# Autodesk Inventor assembly: RT_FRM_A_003_Frame
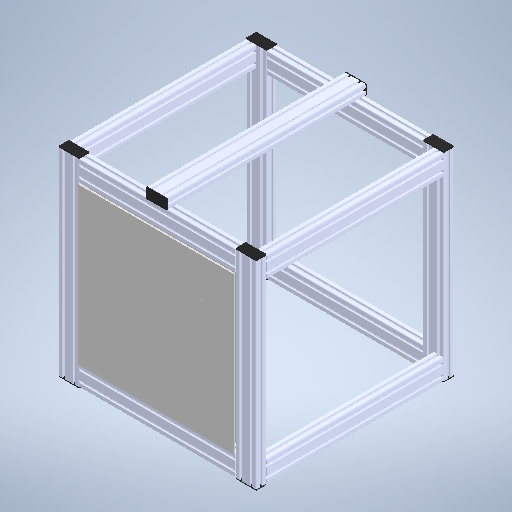
[picture p0: Inventor's stored thumbnail of the model, 512x512]
Saved by Autodesk Inventor 2025.4 (Build 294407000, 407)
## iProperties
Created: 2026-05-11
Part Number: RT_FRM_A_003_Frame
Document SubType Name: Assembly
Designer: louis
Author: louis
## Documents named in this file (7)
- C:\Users\louis\OneDrive\Desktop\R_Trident\02_CAD\04_Subassemblies\RT_FRM_A_003_Frame.iam
- C:\Users\louis\OneDrive\Desktop\R_Trident\02_CAD\01_Standard_Parts\Aluminium_Extrusions\4080x600_3620_2025012844725.ipt
- C:\Users\louis\OneDrive\Desktop\R_Trident\02_CAD\01_Standard_Parts\Aluminium_Extrusions\4080x680_3620_2025012844725.ipt
- C:\Users\louis\OneDrive\Desktop\R_Trident\02_CAD\01_Standard_Parts\Aluminium_Extrusions\4080x760_3620_2025012844725.ipt
- C:\Users\louis\OneDrive\Desktop\R_Trident\02_CAD\01_Standard_Parts\Aluminium_Extrusions\4080-cover.ipt
- C:\Users\louis\OneDrive\Desktop\R_Trident\02_CAD\03_Parts_Custom\RT_FRM_MC_009_ElectricalBackPlate.ipt
- C:\Users\louis\OneDrive\Desktop\R_Trident\02_CAD\03_Parts_Custom\RT_FRM_MC_009_ElectricalBackPlate_Inside.ipt
## Components (28 placed, 6 different names)
1. RT_FRM_MC_009_ElectricalBackPlate:1 — Mate:50, Mate:51, Mate:52
2. RT_FRM_MC_009_ElectricalBackPlate_Inside:1 — Mate:48, Mate:49, Flush:48
3. 4080x680_3620_2025012844725:4 — Mate:10, Mate:11, Flush:14
4. 4080x680_3620_2025012844725:3 — Mate:15, Mate:16, Flush:19
5. 4080x680_3620_2025012844725:2 — Flush:15, Mate:12, Mate:13
6. 4080x680_3620_2025012844725:1 — Mate:17, Mate:18, Flush:20
7. 4080x600_3620_2025012844725:4 — Flush:13, Mate:6, Mate:7
8. 4080x600_3620_2025012844725:3 — Flush:12, Mate:8, Mate:9
9. 4080x600_3620_2025012844725:2 — Mate:4, Mate:5, Flush:11, Mate:50, Mate:52
10. 4080x600_3620_2025012844725:1 — Mate:1, Mate:2, Flush:10, Mate:3, Mate:19, Mate:20, Flush:21, Flush:22, Mate:49, Flush:48
11. 4080x760_3620_2025012844725:5 — Mate:19, Flush:21, Mate:37, Mate:38, Mate:43, Mate:44, Mate:45
12. 4080-cover:6 — Mate:37, Mate:38
13. 4080-cover:11 — Mate:43, Mate:44
14. 4080x760_3620_2025012844725:6 — Mate:20, Flush:22, Mate:39, Mate:40, Mate:41, Mate:42
15. 4080-cover:7 — Mate:39, Mate:40
16. 4080-cover:9 — Mate:41, Mate:42
17. 4080x760_3620_2025012844725:1 — Flush:1, Flush:6, Flush:8, Mate:3, Mate:5, Mate:10, Mate:13, Flush:17, Mate:23, Mate:24, Mate:29, Mate:30, Mate:51
18. 4080-cover:1 — Mate:23, Mate:24
19. 4080-cover:12 — Mate:29, Mate:30
20. 4080x760_3620_2025012844725:2 — Flush:3, Flush:5, Flush:9, Flush:12, Mate:7, Mate:8, Mate:16, Flush:19, Mate:17, Mate:27, Mate:28, Mate:33, Mate:34
21. 4080-cover:5 — Mate:33, Mate:34
22. 4080-cover:10 — Mate:27, Mate:28
23. 4080x760_3620_2025012844725:3 — Flush:2, Flush:6, Flush:9, Flush:13, Mate:6, Mate:9, Mate:11, Flush:14, Flush:15, Mate:12, Flush:16, Mate:25, Mate:26, Mate:35, Mate:36
24. 4080-cover:2 — Mate:35, Mate:36
25. 4080-cover:8 — Mate:25, Mate:26
26. 4080x760_3620_2025012844725:4 — Flush:4, Flush:5, Flush:8, Mate:1, Mate:2, Flush:10, Mate:4, Flush:11, Mate:15, Mate:18, Flush:20, Mate:21, Mate:22, Mate:31, Mate:32, Mate:48
27. 4080-cover:3 — Mate:21, Mate:22
28. 4080-cover:4 — Mate:31, Mate:32
## Relationships (72: Mate 50, Flush 22)
- Flush:1: 4080x760_3620_2025012844725:1
- Flush:2: 4080x760_3620_2025012844725:3
- Flush:3: 4080x760_3620_2025012844725:2
- Flush:4: 4080x760_3620_2025012844725:4
- Flush:5: 4080x760_3620_2025012844725:2 ↔ 4080x760_3620_2025012844725:4
- Flush:6: 4080x760_3620_2025012844725:1 ↔ 4080x760_3620_2025012844725:3
- Flush:8: 4080x760_3620_2025012844725:1 ↔ 4080x760_3620_2025012844725:4
- Flush:9: 4080x760_3620_2025012844725:2 ↔ 4080x760_3620_2025012844725:3
- Mate:1: 4080x600_3620_2025012844725:1 ↔ 4080x760_3620_2025012844725:4
- Mate:2: 4080x600_3620_2025012844725:1 ↔ 4080x760_3620_2025012844725:4
- Flush:10: 4080x600_3620_2025012844725:1 ↔ 4080x760_3620_2025012844725:4
- Mate:3: 4080x600_3620_2025012844725:1 ↔ 4080x760_3620_2025012844725:1
- Mate:4: 4080x600_3620_2025012844725:2 ↔ 4080x760_3620_2025012844725:4
- Mate:5: 4080x600_3620_2025012844725:2 ↔ 4080x760_3620_2025012844725:1
- Flush:11: 4080x600_3620_2025012844725:2 ↔ 4080x760_3620_2025012844725:4
- Flush:12: 4080x600_3620_2025012844725:3 ↔ 4080x760_3620_2025012844725:2
- Flush:13: 4080x600_3620_2025012844725:4 ↔ 4080x760_3620_2025012844725:3
- Mate:6: 4080x600_3620_2025012844725:4 ↔ 4080x760_3620_2025012844725:3
- Mate:7: 4080x600_3620_2025012844725:4 ↔ 4080x760_3620_2025012844725:2
- Mate:8: 4080x600_3620_2025012844725:3 ↔ 4080x760_3620_2025012844725:2
- Mate:9: 4080x600_3620_2025012844725:3 ↔ 4080x760_3620_2025012844725:3
- Mate:10: 4080x680_3620_2025012844725:4 ↔ 4080x760_3620_2025012844725:1
- Mate:11: 4080x680_3620_2025012844725:4 ↔ 4080x760_3620_2025012844725:3
- Flush:14: 4080x680_3620_2025012844725:4 ↔ 4080x760_3620_2025012844725:3
- Flush:15: 4080x680_3620_2025012844725:2 ↔ 4080x760_3620_2025012844725:3
- Mate:12: 4080x680_3620_2025012844725:2 ↔ 4080x760_3620_2025012844725:3
- Mate:13: 4080x680_3620_2025012844725:2 ↔ 4080x760_3620_2025012844725:1
- Flush:16 (-380 mm): 4080x760_3620_2025012844725:3
- Flush:17 (-380 mm): 4080x760_3620_2025012844725:1
- Mate:14
- Flush:18
- Mate:15: 4080x680_3620_2025012844725:3 ↔ 4080x760_3620_2025012844725:4
- Mate:16: 4080x680_3620_2025012844725:3 ↔ 4080x760_3620_2025012844725:2
- Flush:19: 4080x680_3620_2025012844725:3 ↔ 4080x760_3620_2025012844725:2
- Mate:17: 4080x680_3620_2025012844725:1 ↔ 4080x760_3620_2025012844725:2
- Mate:18: 4080x680_3620_2025012844725:1 ↔ 4080x760_3620_2025012844725:4
- Flush:20: 4080x680_3620_2025012844725:1 ↔ 4080x760_3620_2025012844725:4
- Mate:19: 4080x600_3620_2025012844725:1 ↔ 4080x760_3620_2025012844725:5
- Mate:20: 4080x600_3620_2025012844725:1 ↔ 4080x760_3620_2025012844725:6
- Flush:21: 4080x600_3620_2025012844725:1 ↔ 4080x760_3620_2025012844725:5
- Flush:22: 4080x600_3620_2025012844725:1 ↔ 4080x760_3620_2025012844725:6
- Mate:21: 4080x760_3620_2025012844725:4 ↔ 4080-cover:3
- Mate:22: 4080x760_3620_2025012844725:4 ↔ 4080-cover:3
- Mate:23: 4080x760_3620_2025012844725:1 ↔ 4080-cover:1
- Mate:24: 4080x760_3620_2025012844725:1 ↔ 4080-cover:1
- Mate:25: 4080x760_3620_2025012844725:3 ↔ 4080-cover:8
- Mate:26: 4080x760_3620_2025012844725:3 ↔ 4080-cover:8
- Mate:27: 4080x760_3620_2025012844725:2 ↔ 4080-cover:10
- Mate:28: 4080x760_3620_2025012844725:2 ↔ 4080-cover:10
- Mate:29: 4080x760_3620_2025012844725:1 ↔ 4080-cover:12
- Mate:30: 4080x760_3620_2025012844725:1 ↔ 4080-cover:12
- Mate:31: 4080x760_3620_2025012844725:4 ↔ 4080-cover:4
- Mate:32: 4080x760_3620_2025012844725:4 ↔ 4080-cover:4
- Mate:33: 4080x760_3620_2025012844725:2 ↔ 4080-cover:5
- Mate:34: 4080x760_3620_2025012844725:2 ↔ 4080-cover:5
- Mate:35: 4080x760_3620_2025012844725:3 ↔ 4080-cover:2
- Mate:36: 4080x760_3620_2025012844725:3 ↔ 4080-cover:2
- Mate:37: 4080x760_3620_2025012844725:5 ↔ 4080-cover:6
- Mate:38: 4080x760_3620_2025012844725:5 ↔ 4080-cover:6
- Mate:39: 4080x760_3620_2025012844725:6 ↔ 4080-cover:7
- Mate:40: 4080x760_3620_2025012844725:6 ↔ 4080-cover:7
- Mate:41: 4080x760_3620_2025012844725:6 ↔ 4080-cover:9
- Mate:42: 4080x760_3620_2025012844725:6 ↔ 4080-cover:9
- Mate:43: 4080x760_3620_2025012844725:5 ↔ 4080-cover:11
- Mate:44: 4080x760_3620_2025012844725:5 ↔ 4080-cover:11
- Mate:45 (-40 mm): 4080x760_3620_2025012844725:5
- Mate:48: RT_FRM_MC_009_ElectricalBackPlate_Inside:1 ↔ 4080x760_3620_2025012844725:4
- Mate:49: RT_FRM_MC_009_ElectricalBackPlate_Inside:1 ↔ 4080x600_3620_2025012844725:1
- Flush:48: RT_FRM_MC_009_ElectricalBackPlate_Inside:1 ↔ 4080x600_3620_2025012844725:1
- Mate:50: RT_FRM_MC_009_ElectricalBackPlate:1 ↔ 4080x600_3620_2025012844725:2
- Mate:51: RT_FRM_MC_009_ElectricalBackPlate:1 ↔ 4080x760_3620_2025012844725:1
- Mate:52: RT_FRM_MC_009_ElectricalBackPlate:1 ↔ 4080x600_3620_2025012844725:2
